# Autodesk Inventor assembly: Общая сборка
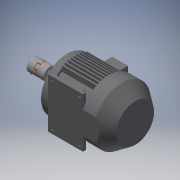
[picture p0: Inventor's stored thumbnail of the model, 180x180]
Saved by Autodesk Inventor 2016 (Build 200138000, 138)
## iProperties
Created: 2021-04-30
Part Number: Общая сборка
Material: Типовые
Document SubType Name: Assembly
Designer: Лол
Author: Лол
## Documents named in this file (3)
- C:\Users\Лол\Documents\Inventor\course_work\Общая сборка.iam
- C:\Users\Лол\Documents\Inventor\course_work\Муфта двигателя.iam
- C:\Users\Лол\Documents\Inventor\course_work\Электродвигатель АИР132S4,6,8.ipt
## Components (2 placed, 2 different names)
1. Муфта двигателя:1 [sub-assembly] — Совмещение:1, Совмещение:2, Совмещение:3
2. Электродвигатель АИР132S4,6,8:1 — Совмещение:1, Совмещение:2, Совмещение:3
## Relationships (3: Mate 3)
- Совмещение:1 [Mate]: Муфта двигателя:1 ↔ Электродвигатель АИР132S4,6,8:1
- Совмещение:2 [Mate]: Муфта двигателя:1 ↔ Электродвигатель АИР132S4,6,8:1
- Совмещение:3 [Mate] (-30 mm): Муфта двигателя:1 ↔ Электродвигатель АИР132S4,6,8:1
